# Autodesk Inventor assembly: 200-03-BOGIE-CONNECTOR-ASM
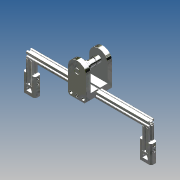
[picture p0: Inventor's stored thumbnail of the model, 180x180]
Saved by Autodesk Inventor 2018.2 (Build 222227000, 227)
## iProperties
Manager: feesmrt
Company: FRANC0R
Created: 2017-12-19
Part Number: 200-03-BOGIE-CONNECTOR-ASM
Project: Rescue Robot
Cost Center: -
Material: Generisch
Document SubType Name: Assembly
Designer: feesmrt
Engineer: feesmrt
Authority: feesmrt
Description: Bogie Connector
Stock Number: 200-03-BOGIE-CONNECTOR-ASM-L
Subject: Rescue Robot
Author: feesmrt
Revision Number: 1
Title: Bogie Connector
## Documents named in this file (3)
- D:\Programmierung\FRANC0R\CAD\02-Rocker-Bogie-Robot\200-ROCKER-BOGIE\200-03-BOGIE-CONNECTOR-ASM.iam
- D:\Programmierung\FRANC0R\CAD\02-Rocker-Bogie-Robot\200-ROCKER-BOGIE\200-40-BOGIE-CONNECTOR\200-40-BOGIE-CONNECTOR-ASM-01.iam
- D:\Programmierung\FRANC0R\CAD\02-Rocker-Bogie-Robot\200-ROCKER-BOGIE\200-50-WHEEL-CONNECTOR\200-50-WHEEL-CONNECTOR-20MM-ASM-01.iam
## Components (3 placed, 2 different names)
1. 200-40-BOGIE-CONNECTOR-ASM-01:1 [sub-assembly] — Passend:1, Passend:2, Fluchtend:1, Passend:3, Fluchtend:2, Passend:4
2. 200-50-WHEEL-CONNECTOR-20MM-ASM-01:1 [sub-assembly] — Passend:1, Passend:2, Fluchtend:1
3. 200-50-WHEEL-CONNECTOR-20MM-ASM-01:2 [sub-assembly] — Passend:3, Fluchtend:2, Passend:4
## Relationships (6: Mate 4, Flush 2)
- Passend:1 [Mate]: 200-40-BOGIE-CONNECTOR-ASM-01:1 ↔ 200-50-WHEEL-CONNECTOR-20MM-ASM-01:1
- Passend:2 [Mate]: 200-40-BOGIE-CONNECTOR-ASM-01:1 ↔ 200-50-WHEEL-CONNECTOR-20MM-ASM-01:1
- Fluchtend:1 [Flush]: 200-40-BOGIE-CONNECTOR-ASM-01:1 ↔ 200-50-WHEEL-CONNECTOR-20MM-ASM-01:1
- Passend:3 [Mate]: 200-40-BOGIE-CONNECTOR-ASM-01:1 ↔ 200-50-WHEEL-CONNECTOR-20MM-ASM-01:2
- Fluchtend:2 [Flush]: 200-40-BOGIE-CONNECTOR-ASM-01:1 ↔ 200-50-WHEEL-CONNECTOR-20MM-ASM-01:2
- Passend:4 [Mate]: 200-40-BOGIE-CONNECTOR-ASM-01:1 ↔ 200-50-WHEEL-CONNECTOR-20MM-ASM-01:2
